# Autodesk Inventor assembly: PrinterMini
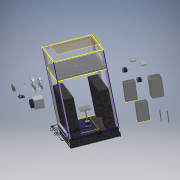
[picture p0: Inventor's stored thumbnail of the model, 180x180]
Saved by Autodesk Inventor 2016 (Build 200138000, 138)
## iProperties
Created: 2015-08-01
Part Number: PrinterMini
Document SubType Name: Assembly
Designer: myhome
Author: myhome
## Documents named in this file (15)
- C:\Users\myhome\Documents\Inventor\Printer\PrinterMini.iam
- C:\Users\myhome\Documents\Inventor\Printer\EpoxyGraniteBase\BaseMini.iam
- C:\Users\myhome\Documents\Inventor\Printer\FrameExtruded\FrameMini.iam
- C:\Users\myhome\Documents\Inventor\Printer\FrameSheetMetal\FrameSheetLaserViewportMini.ipt
- C:\Users\myhome\Documents\Inventor\Printer\SilverstoneFan\SilverstoneFQ121.iam
- C:\Users\myhome\Documents\Inventor\Printer\RaspberryPiCamera\RaspberryPiCamera.ipt
- C:\Users\myhome\Documents\Inventor\Printer\RaspberryPi2\RaspberryPi2.iam
- C:\Users\myhome\Documents\Inventor\Printer\GShield\GShield.iam
- C:\Users\myhome\Documents\Inventor\Printer\ScanCube\WarpCube.iam
- C:\Users\myhome\Documents\Inventor\Printer\Nema17Motor\Nema17Stepper.iam
- C:\Users\myhome\Documents\Inventor\Printer\PistonHead\PistonFeederHeadMini.iam
- C:\Users\myhome\Documents\Inventor\Printer\PistonHead\PistonWorkHeadMini.iam
- C:\Users\myhome\Documents\Inventor\Printer\PistonFrame\PistonFeederFrameMini.iam
- C:\Users\myhome\Documents\Inventor\Printer\PistonFrame\PistonWorkFrameMini.iam
- C:\Users\myhome\Documents\Inventor\Printer\LinearActuator\LinearActuatorMini.iam
## Components (21 placed, 14 different names)
1. BaseMini:1 [sub-assembly] — Mate:3, Mate:4, Rigid:2
2. FrameMini:1 [sub-assembly] — Mate:3, Mate:4, Mate:5, Mate:6
3. FrameSheetLaserViewportMini:1 — Mate:5, Mate:6
4. SilverstoneFQ121:2 [sub-assembly]
5. SilverstoneFQ121:3 [sub-assembly]
6. RaspberryPiCamera:1
7. RaspberryPi2:1 [sub-assembly]
8. GShield:1 [sub-assembly]
9. WarpCube:1 [sub-assembly]
10. Nema17Stepper:1 [sub-assembly]
11. Nema17Stepper:2 [sub-assembly]
12. Nema17Stepper:3 [sub-assembly] — Rotational:1, Rigid:2
13. PistonFeederHeadMini:1 [sub-assembly]
14. PistonFeederHeadMini:2 [sub-assembly]
15. PistonWorkHeadMini:1 [sub-assembly] — Rigid:1
16. PistonFrameMini:1 [sub-assembly]
17. PistonFrameMini:2 [sub-assembly]
18. PistonWorkFrameMini:1 [sub-assembly]
19. LinearActuatorMini:1 [sub-assembly] — Rotational:1, Rigid:1
20. LinearActuatorMini:2 [sub-assembly]
21. LinearActuatorMini:3 [sub-assembly]
## Relationships (7: Mate 4, WeldJoint 2, RevoluteJoint 1)
- Mate:3: BaseMini:1 ↔ FrameMini:1
- Mate:4: BaseMini:1 ↔ FrameMini:1
- Mate:5: FrameMini:1 ↔ FrameSheetLaserViewportMini:1
- Mate:6: FrameMini:1 ↔ FrameSheetLaserViewportMini:1
- Rotational:1 [RevoluteJoint]: Nema17Stepper:3 ↔ LinearActuatorMini:1
- Rigid:1 [WeldJoint]: PistonWorkHeadMini:1 ↔ LinearActuatorMini:1
- Rigid:2 [WeldJoint]: BaseMini:1 ↔ Nema17Stepper:3
